# Autodesk Inventor assembly: Lager
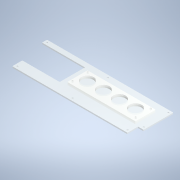
[picture p0: Inventor's stored thumbnail of the model, 180x180]
Saved by Autodesk Inventor 2022 (Build 260153000, 153)
## iProperties
Created: 2021-12-01
Part Number: Lager
Document SubType Name: Assembly
Designer: Fabijan_Sven
Author: Fabijan_Sven
## Documents named in this file (4)
- E:\Transfer\Sync\Hivemind\1-MCI-Unterlagen\Master\Semester 3\Projekt 2\011_Kartesischer_Roboter_Modul\07-CAD Files\05-Lager\Lager.iam
- E:\Transfer\Sync\Hivemind\1-MCI-Unterlagen\Master\Semester 3\Projekt 2\011_Kartesischer_Roboter_Modul\07-CAD Files\05-Lager\BasePlate.ipt
- E:\Transfer\Sync\Hivemind\1-MCI-Unterlagen\Master\Semester 3\Projekt 2\011_Kartesischer_Roboter_Modul\07-CAD Files\05-Lager\HolePlates.ipt
- E:\Transfer\Sync\Hivemind\1-MCI-Unterlagen\Master\Semester 3\Projekt 2\011_Kartesischer_Roboter_Modul\07-CAD Files\05-Lager\ClosedPlates.ipt
## Components (3 placed, 3 different names)
1. BasePlate:1 — Mate:1, Mate:3, Mate:4
2. HolePlates:1 — Mate:1, Mate:3, Mate:4, Mate:5, Mate:6, Mate:7
3. ClosedPlates:1 — Mate:5, Mate:6, Mate:7
## Relationships (6: Mate 6)
- Mate:1: BasePlate:1 ↔ HolePlates:1
- Mate:3: BasePlate:1 ↔ HolePlates:1
- Mate:4: BasePlate:1 ↔ HolePlates:1
- Mate:5: HolePlates:1 ↔ ClosedPlates:1
- Mate:6: HolePlates:1 ↔ ClosedPlates:1
- Mate:7: HolePlates:1 ↔ ClosedPlates:1
